# Autodesk Inventor assembly: Y_Slider_mit_Schrittmotor
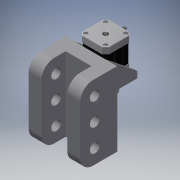
[picture p0: Inventor's stored thumbnail of the model, 180x180]
Saved by Autodesk Inventor 2019 (Build 230136000, 136)
## iProperties
Created: 2018-08-24
Part Number: Y_Slider_mit_Schrittmotor
Document SubType Name: Assembly
Designer: Julia
Author: Julia
## Documents named in this file (5)
- C:\Users\Julia\Documents\Inventor\3d_Drucker_v03_vertikaler_Gurt\Y_Slider_mit_Schrittmotor.iam
- C:\Users\Julia\Documents\Inventor\3d_Drucker_v03_vertikaler_Gurt\Schrittmotor_Nema_17.ipt
- C:\Users\Julia\Documents\Inventor\3d_Drucker_v03_vertikaler_Gurt\Metallstange_Slider.ipt
- C:\Users\Julia\Documents\Inventor\3d_Drucker_v03_vertikaler_Gurt\Y_Slider_Zahnrad.ipt
- C:\Users\Julia\Documents\Inventor\3d_Drucker_v03_vertikaler_Gurt\Y_Slider_Part_mit_Schrittmotor.ipt
## Components (7 placed, 4 different names)
1. Schrittmotor_Nema_17:1 — Mate:8, Mate:9, Mate:10, Mate:11
2. Metallstange_Slider:1 — Mate:13, Flush:1
3. Metallstange_Slider:2 — Mate:14, Flush:2
4. Metallstange_Slider:3 — Mate:16, Flush:3
5. Metallstange_Slider:4 — Mate:15, Flush:4
6. Y_Slider_Zahnrad:1 — Mate:8, Mate:12
7. Y_Slider_Part_mit_Schrittmotor:1 — Mate:9, Mate:10, Mate:11, Mate:12, Mate:13, Mate:14, Flush:1, Flush:2, Mate:15, Mate:16, Flush:3, Flush:4
## Relationships (13: Mate 9, Flush 4)
- Mate:8: Schrittmotor_Nema_17:1 ↔ Y_Slider_Zahnrad:1
- Mate:9: Schrittmotor_Nema_17:1 ↔ Y_Slider_Part_mit_Schrittmotor:1
- Mate:10: Schrittmotor_Nema_17:1 ↔ Y_Slider_Part_mit_Schrittmotor:1
- Mate:11: Schrittmotor_Nema_17:1 ↔ Y_Slider_Part_mit_Schrittmotor:1
- Mate:12 (3 mm): Y_Slider_Zahnrad:1 ↔ Y_Slider_Part_mit_Schrittmotor:1
- Mate:13: Metallstange_Slider:1 ↔ Y_Slider_Part_mit_Schrittmotor:1
- Mate:14: Metallstange_Slider:2 ↔ Y_Slider_Part_mit_Schrittmotor:1
- Flush:1: Metallstange_Slider:1 ↔ Y_Slider_Part_mit_Schrittmotor:1
- Flush:2: Metallstange_Slider:2 ↔ Y_Slider_Part_mit_Schrittmotor:1
- Mate:15: Metallstange_Slider:4 ↔ Y_Slider_Part_mit_Schrittmotor:1
- Mate:16: Metallstange_Slider:3 ↔ Y_Slider_Part_mit_Schrittmotor:1
- Flush:3: Metallstange_Slider:3 ↔ Y_Slider_Part_mit_Schrittmotor:1
- Flush:4: Metallstange_Slider:4 ↔ Y_Slider_Part_mit_Schrittmotor:1
